# Autodesk Inventor assembly: Shooter
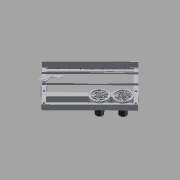
[picture p0: Inventor's stored thumbnail of the model, 180x180]
Saved by Autodesk Inventor 2013 (Build 170138000, 138)
## iProperties
Created: 2013-01-27
Part Number: Shooter
Document SubType Name: Assembly
Designer: Naphat
Author: Naphat
## Documents named in this file (19)
- C:\Autodesk\gruntmaster6000-cad\Shooter6000-cad\Shooter\Shooter.iam
- C:\Autodesk\gruntmaster6000-cad\Shooter6000-cad\Shooter\Basic Wheel\Shooter Basic Design.iam
- C:\Autodesk\gruntmaster6000-cad\Shooter6000-cad\Shooter\26in Angle Channel.ipt
- C:\Autodesk\gruntmaster6000-cad\Shooter6000-cad\Shooter\26in mini C-Channel (rail).ipt
- C:\Users\Naphat\Documents\Inventor\Content Center Files\R2013\en-US\ANSI B18.3(05)\ANSI B18.3 - 1_4-20 UNC - 1(31).ipt
- C:\Users\Naphat\Documents\Inventor\Content Center Files\R2013\en-US\ASTM F436(1)\ASTM F436 - 1_4(1).ipt
- C:\Users\Naphat\Documents\Inventor\Content Center Files\R2013\en-US\IFI 100 107(2)\IFI 100_107 - 1_4 - 20 Metal Type.ipt
- C:\Autodesk\gruntmaster6000-cad\Shooter6000-cad\Shooter\18in C-Channel Front.ipt
- C:\Autodesk\gruntmaster6000-cad\Shooter6000-cad\Shooter\18in C-Channel Rear.ipt
- C:\Users\Naphat\Documents\Inventor\Content Center Files\R2013\en-US\ANSI B18.3(05)\ANSI B18.3 - 1_4-20 UNC - 1.75(31).ipt
- C:\Autodesk\gruntmaster6000-cad\Shooter6000-cad\Shooter\26in Angle Channel CIM Mount Left.ipt
- C:\Autodesk\gruntmaster6000-cad\Shooter6000-cad\Shooter\26in Angle Channel CIM Mount Right.ipt
- C:\Autodesk\gruntmaster6000-cad\Shooter6000-cad\Shooter\26in C-Channel Left.ipt
- C:\Autodesk\gruntmaster6000-cad\Shooter6000-cad\Shooter\26in C-Channel Right.ipt
- C:\Autodesk\gruntmaster6000-cad\Shooter6000-cad\Shooter\Motors\CIM Case\CIM Mount Bolt.ipt
- C:\Autodesk\gruntmaster6000-cad\Shooter6000-cad\Shooter\Firing Pin\Firing Pin.iam
- C:\Autodesk\gruntmaster6000-cad\Shooter6000-cad\Shooter\Frisbee.ipt
- C:\Autodesk\gruntmaster6000-cad\Shooter6000-cad\Imported Components\PG27\PG27.ipt
- C:\Users\Naphat\Documents\Inventor\Content Center Files\R2013\en-US\IFI 100 107(2)\IFI 100_107 - 1_4 - 20 Top Insert Type.ipt
## Components (62 placed, 18 different names)
1. Shooter Basic Design:1 [sub-assembly] — Insert:2, Insert:3
2. Shooter Basic Design:2 [sub-assembly] — Insert:4, Insert:5
3. 26in C-Channel Right:1 — Flush:3, Mate:1, Mate:2, Mate:5, Mate:7, Flush:5, Mate:156, Insert:6, Insert:7, Insert:16, Mate:220, Mate:221
4. 18in C-Channel Rear — Flush:3, Mate:1, Mate:2, Flush:4, Mate:3, Mate:4, Flush:9, Mate:82, Mate:207, Mate:208, Mate:212, Mate:214, Insert:8
5. 18in C-Channel Front — Mate:5, Mate:6, Mate:7, Flush:5, Flush:12, Mate:23, Flush:13, Mate:24, Flush:14, Mate:74, Mate:213, Insert:13
6. 26in C-Channel Left:1 — Flush:4, Mate:3, Mate:4, Mate:6, Mate:8, Mate:9, Mate:75, Mate:76, Mate:77, Mate:78, Mate:79, Mate:80, Mate:81
7. 26in Angle Channel:1 — Mate:8, Mate:9, Flush:9, Mate:25, Mate:36, Mate:38, Mate:39, Mate:40, Mate:41, Mate:42, Mate:43, Mate:44, Mate:45, Mate:46, Mate:47, Mate:48, Mate:49, Mate:50, Mate:51, Mate:52, Mate:53, Mate:54, Mate:55, Mate:56, Mate:57, Mate:58, Mate:59, Mate:60, Mate:61, Mate:62, Mate:63
8. 26in Angle Channel CIM Mount Right:1 — Mate:189, Mate:190, Mate:191, Mate:192, Mate:193, Mate:194, Mate:195, Mate:196, Insert:6, Insert:7, Mate:216, Mate:217, Mate:218, Mate:219
9. 26in Angle Channel CIM Mount Left:3 — Flush:12, Mate:213, Mate:214, Insert:9, Insert:12
10. 26in mini C-Channel (rail):1 — Mate:23, Flush:13, Mate:26, Mate:206
11. 26in mini C-Channel (rail):2 — Mate:24, Flush:14, Mate:25, Mate:26
12. CIM Mount Bolt:1 — Mate:192, Mate:196, Insert:4
13. CIM Mount Bolt:2 — Mate:191, Mate:195, Insert:5
14. CIM Mount Bolt:3 — Mate:189, Mate:193, Insert:2
15. CIM Mount Bolt:4 — Mate:190, Mate:194, Insert:3
16. Firing Pin:1 [sub-assembly] — Mate:207, Mate:208, Mate:210, Mate:211
17. Frisbee:1 — Mate:206
18. PG27:1 — Mate:210, Mate:211, Mate:212
19. Circular Washer (Inch) 1/4:29 — Insert:8, Insert:10
20. Circular Washer (Inch) 1/4:30 — Insert:9, Insert:11
21. Hexagon Socket Head Cap Screw - Inch 1/4 - 20 UNC - 1 3/4:1 — Insert:10, Mate:215
22. Prevailing Torque Type Hex Nut - Inch (IFI) 1/4 - 20 Top Insert Type:1 — Insert:11, Mate:215
23. Circular Washer (Inch) 1/4:31 — Insert:12, Insert:15
24. Circular Washer (Inch) 1/4:32 — Insert:13, Insert:14
25. Hexagon Socket Head Cap Screw - Inch 1/4 - 20 UNC - 1 3/4:2 — Insert:14
26. Prevailing Torque Type Hex Nut - Inch (IFI) 1/4 - 20 Top Insert Type:2 — Insert:15
27. Circular Washer (Inch) 1/4:33 — Insert:16, Mate:222, Mate:223
28. Circular Washer (Inch) 1/4:34 — Mate:216, Mate:217, Mate:226
29. Circular Washer (Inch) 1/4:35 — Mate:218, Mate:219, Mate:228
30. Circular Washer (Inch) 1/4:36 — Mate:220, Mate:221, Mate:224, Mate:225
31. Hexagon Socket Head Cap Screw - Inch 1/4 - 20 UNC - 1 3/4:3 — Mate:224, Mate:225, Mate:229
32. Hexagon Socket Head Cap Screw - Inch 1/4 - 20 UNC - 1 3/4:4 — Mate:222, Mate:223, Mate:227
33. Prevailing Torque Type Hex Nut - Inch (IFI) 1/4 - 20 Top Insert Type:3 — Mate:228, Mate:229
34. Prevailing Torque Type Hex Nut - Inch (IFI) 1/4 - 20 Top Insert Type:4 — Mate:226, Mate:227
35. Hexagon Socket Head Cap Screw - Inch 1/4 - 20 UNC - 1:1 — Mate:36, Mate:72, Mate:91
36. Hexagon Socket Head Cap Screw - Inch 1/4 - 20 UNC - 1:3 — Mate:39, Mate:70, Mate:89
37. Hexagon Socket Head Cap Screw - Inch 1/4 - 20 UNC - 1:4 — Mate:38, Mate:71, Mate:90
38. Hexagon Socket Head Cap Screw - Inch 1/4 - 20 UNC - 1:10 — Mate:43, Mate:66, Mate:85
39. Hexagon Socket Head Cap Screw - Inch 1/4 - 20 UNC - 1:11 — Mate:40, Mate:69, Mate:88
40. Hexagon Socket Head Cap Screw - Inch 1/4 - 20 UNC - 1:14 — Mate:42, Mate:67, Mate:86
41. Hexagon Socket Head Cap Screw - Inch 1/4 - 20 UNC - 1:16 — Mate:44, Mate:65, Mate:84
42. Hexagon Socket Head Cap Screw - Inch 1/4 - 20 UNC - 1:18 — Mate:45, Mate:64, Mate:83
43. Hexagon Socket Head Cap Screw - Inch 1/4 - 20 UNC - 1:22 — Mate:41, Mate:68, Mate:87
44. Prevailing Torque Type Hex Nut - Inch (IFI) 1/4 - 20 Metal Type:2 — Mate:78, Mate:87
45. Prevailing Torque Type Hex Nut - Inch (IFI) 1/4 - 20 Metal Type:8 — Mate:80, Mate:85
46. Prevailing Torque Type Hex Nut - Inch (IFI) 1/4 - 20 Metal Type:9 — Mate:77, Mate:88
47. Prevailing Torque Type Hex Nut - Inch (IFI) 1/4 - 20 Metal Type:14 — Mate:82, Mate:83
48. Prevailing Torque Type Hex Nut - Inch (IFI) 1/4 - 20 Metal Type:24 — Mate:81, Mate:84
49. Prevailing Torque Type Hex Nut - Inch (IFI) 1/4 - 20 Metal Type:27 — Mate:156
50. Prevailing Torque Type Hex Nut - Inch (IFI) 1/4 - 20 Metal Type:41 — Mate:75, Mate:90
51. Prevailing Torque Type Hex Nut - Inch (IFI) 1/4 - 20 Metal Type:42 — Mate:76, Mate:89
52. Prevailing Torque Type Hex Nut - Inch (IFI) 1/4 - 20 Metal Type:43 — Mate:74, Mate:91
53. Prevailing Torque Type Hex Nut - Inch (IFI) 1/4 - 20 Metal Type:48 — Mate:79, Mate:86
54. Circular Washer (Inch) 1/4:1 — Mate:48, Mate:57, Mate:70
55. Circular Washer (Inch) 1/4:2 — Mate:49, Mate:58, Mate:69
56. Circular Washer (Inch) 1/4:3 — Mate:47, Mate:56, Mate:71
57. Circular Washer (Inch) 1/4:4 — Mate:46, Mate:55, Mate:72
58. Circular Washer (Inch) 1/4:7 — Mate:52, Mate:61, Mate:66
59. Circular Washer (Inch) 1/4:8 — Mate:54, Mate:63, Mate:64
60. Circular Washer (Inch) 1/4:9 — Mate:51, Mate:60, Mate:67
61. Circular Washer (Inch) 1/4:10 — Mate:53, Mate:62, Mate:65
62. Circular Washer (Inch) 1/4:28 — Mate:50, Mate:59, Mate:68
## Relationships (121: Mate 99, Insert 15, Flush 7)
- Flush:3: 26in C-Channel Right:1 ↔ 18in C-Channel Rear
- Mate:1: 26in C-Channel Right:1 ↔ 18in C-Channel Rear
- Mate:2: 26in C-Channel Right:1 ↔ 18in C-Channel Rear
- Flush:4: 18in C-Channel Rear ↔ 26in C-Channel Left:1
- Mate:3: 18in C-Channel Rear ↔ 26in C-Channel Left:1
- Mate:4: 18in C-Channel Rear ↔ 26in C-Channel Left:1
- Mate:5: 26in C-Channel Right:1 ↔ 18in C-Channel Front
- Mate:6: 18in C-Channel Front ↔ 26in C-Channel Left:1
- Mate:7: 26in C-Channel Right:1 ↔ 18in C-Channel Front
- Flush:5: 26in C-Channel Right:1 ↔ 18in C-Channel Front
- Mate:8 (-25 mm): 26in C-Channel Left:1 ↔ 26in Angle Channel:1
- Mate:9: 26in C-Channel Left:1 ↔ 26in Angle Channel:1
- Flush:9: 18in C-Channel Rear ↔ 26in Angle Channel:1
- Flush:12: 18in C-Channel Front ↔ 26in Angle Channel CIM Mount Left:3
- Mate:23: 18in C-Channel Front ↔ 26in mini C-Channel (rail):1
- Flush:13: 18in C-Channel Front ↔ 26in mini C-Channel (rail):1
- Mate:24: 18in C-Channel Front ↔ 26in mini C-Channel (rail):2
- Flush:14: 18in C-Channel Front ↔ 26in mini C-Channel (rail):2
- Mate:25 (69.75 mm): 26in Angle Channel:1 ↔ 26in mini C-Channel (rail):2
- Mate:26 (129.5 mm): 26in mini C-Channel (rail):1 ↔ 26in mini C-Channel (rail):2
- Mate:36: 26in Angle Channel:1 ↔ Hexagon Socket Head Cap Screw - Inch 1/4 - 20 UNC - 1:1
- Mate:38: 26in Angle Channel:1 ↔ Hexagon Socket Head Cap Screw - Inch 1/4 - 20 UNC - 1:4
- Mate:39: 26in Angle Channel:1 ↔ Hexagon Socket Head Cap Screw - Inch 1/4 - 20 UNC - 1:3
- Mate:40: 26in Angle Channel:1 ↔ Hexagon Socket Head Cap Screw - Inch 1/4 - 20 UNC - 1:11
- Mate:41: 26in Angle Channel:1 ↔ Hexagon Socket Head Cap Screw - Inch 1/4 - 20 UNC - 1:22
- Mate:42: 26in Angle Channel:1 ↔ Hexagon Socket Head Cap Screw - Inch 1/4 - 20 UNC - 1:14
- Mate:43: 26in Angle Channel:1 ↔ Hexagon Socket Head Cap Screw - Inch 1/4 - 20 UNC - 1:10
- Mate:44: 26in Angle Channel:1 ↔ Hexagon Socket Head Cap Screw - Inch 1/4 - 20 UNC - 1:16
- Mate:45: 26in Angle Channel:1 ↔ Hexagon Socket Head Cap Screw - Inch 1/4 - 20 UNC - 1:18
- Mate:46: 26in Angle Channel:1 ↔ Circular Washer (Inch) 1/4:4
- Mate:47: 26in Angle Channel:1 ↔ Circular Washer (Inch) 1/4:3
- Mate:48: 26in Angle Channel:1 ↔ Circular Washer (Inch) 1/4:1
- Mate:49: 26in Angle Channel:1 ↔ Circular Washer (Inch) 1/4:2
- Mate:50: 26in Angle Channel:1 ↔ Circular Washer (Inch) 1/4:28
- Mate:51: 26in Angle Channel:1 ↔ Circular Washer (Inch) 1/4:9
- Mate:52: 26in Angle Channel:1 ↔ Circular Washer (Inch) 1/4:7
- Mate:53: 26in Angle Channel:1 ↔ Circular Washer (Inch) 1/4:10
- Mate:54: 26in Angle Channel:1 ↔ Circular Washer (Inch) 1/4:8
- Mate:55: 26in Angle Channel:1 ↔ Circular Washer (Inch) 1/4:4
- Mate:56: 26in Angle Channel:1 ↔ Circular Washer (Inch) 1/4:3
- Mate:57: 26in Angle Channel:1 ↔ Circular Washer (Inch) 1/4:1
- Mate:58: 26in Angle Channel:1 ↔ Circular Washer (Inch) 1/4:2
- Mate:59: 26in Angle Channel:1 ↔ Circular Washer (Inch) 1/4:28
- Mate:60: 26in Angle Channel:1 ↔ Circular Washer (Inch) 1/4:9
- Mate:61: 26in Angle Channel:1 ↔ Circular Washer (Inch) 1/4:7
- Mate:62: 26in Angle Channel:1 ↔ Circular Washer (Inch) 1/4:10
- Mate:63: 26in Angle Channel:1 ↔ Circular Washer (Inch) 1/4:8
- Mate:64: Hexagon Socket Head Cap Screw - Inch 1/4 - 20 UNC - 1:18 ↔ Circular Washer (Inch) 1/4:8
- Mate:65: Hexagon Socket Head Cap Screw - Inch 1/4 - 20 UNC - 1:16 ↔ Circular Washer (Inch) 1/4:10
- Mate:66: Hexagon Socket Head Cap Screw - Inch 1/4 - 20 UNC - 1:10 ↔ Circular Washer (Inch) 1/4:7
- Mate:67: Hexagon Socket Head Cap Screw - Inch 1/4 - 20 UNC - 1:14 ↔ Circular Washer (Inch) 1/4:9
- Mate:68: Hexagon Socket Head Cap Screw - Inch 1/4 - 20 UNC - 1:22 ↔ Circular Washer (Inch) 1/4:28
- Mate:69: Hexagon Socket Head Cap Screw - Inch 1/4 - 20 UNC - 1:11 ↔ Circular Washer (Inch) 1/4:2
- Mate:70: Hexagon Socket Head Cap Screw - Inch 1/4 - 20 UNC - 1:3 ↔ Circular Washer (Inch) 1/4:1
- Mate:71: Hexagon Socket Head Cap Screw - Inch 1/4 - 20 UNC - 1:4 ↔ Circular Washer (Inch) 1/4:3
- Mate:72: Hexagon Socket Head Cap Screw - Inch 1/4 - 20 UNC - 1:1 ↔ Circular Washer (Inch) 1/4:4
- Mate:74: 18in C-Channel Front ↔ Prevailing Torque Type Hex Nut - Inch (IFI) 1/4 - 20 Metal Type:43
- Mate:75: 26in C-Channel Left:1 ↔ Prevailing Torque Type Hex Nut - Inch (IFI) 1/4 - 20 Metal Type:41
- Mate:76: 26in C-Channel Left:1 ↔ Prevailing Torque Type Hex Nut - Inch (IFI) 1/4 - 20 Metal Type:42
- Mate:77: 26in C-Channel Left:1 ↔ Prevailing Torque Type Hex Nut - Inch (IFI) 1/4 - 20 Metal Type:9
- Mate:78: 26in C-Channel Left:1 ↔ Prevailing Torque Type Hex Nut - Inch (IFI) 1/4 - 20 Metal Type:2
- Mate:79: 26in C-Channel Left:1 ↔ Prevailing Torque Type Hex Nut - Inch (IFI) 1/4 - 20 Metal Type:48
- Mate:80: 26in C-Channel Left:1 ↔ Prevailing Torque Type Hex Nut - Inch (IFI) 1/4 - 20 Metal Type:8
- Mate:81: 26in C-Channel Left:1 ↔ Prevailing Torque Type Hex Nut - Inch (IFI) 1/4 - 20 Metal Type:24
- Mate:82: 18in C-Channel Rear ↔ Prevailing Torque Type Hex Nut - Inch (IFI) 1/4 - 20 Metal Type:14
- Mate:83: Hexagon Socket Head Cap Screw - Inch 1/4 - 20 UNC - 1:18 ↔ Prevailing Torque Type Hex Nut - Inch (IFI) 1/4 - 20 Metal Type:14
- Mate:84: Hexagon Socket Head Cap Screw - Inch 1/4 - 20 UNC - 1:16 ↔ Prevailing Torque Type Hex Nut - Inch (IFI) 1/4 - 20 Metal Type:24
- Mate:85: Hexagon Socket Head Cap Screw - Inch 1/4 - 20 UNC - 1:10 ↔ Prevailing Torque Type Hex Nut - Inch (IFI) 1/4 - 20 Metal Type:8
- Mate:86: Hexagon Socket Head Cap Screw - Inch 1/4 - 20 UNC - 1:14 ↔ Prevailing Torque Type Hex Nut - Inch (IFI) 1/4 - 20 Metal Type:48
- Mate:87: Hexagon Socket Head Cap Screw - Inch 1/4 - 20 UNC - 1:22 ↔ Prevailing Torque Type Hex Nut - Inch (IFI) 1/4 - 20 Metal Type:2
- Mate:88: Hexagon Socket Head Cap Screw - Inch 1/4 - 20 UNC - 1:11 ↔ Prevailing Torque Type Hex Nut - Inch (IFI) 1/4 - 20 Metal Type:9
- Mate:89: Hexagon Socket Head Cap Screw - Inch 1/4 - 20 UNC - 1:3 ↔ Prevailing Torque Type Hex Nut - Inch (IFI) 1/4 - 20 Metal Type:42
- Mate:90: Hexagon Socket Head Cap Screw - Inch 1/4 - 20 UNC - 1:4 ↔ Prevailing Torque Type Hex Nut - Inch (IFI) 1/4 - 20 Metal Type:41
- Mate:91: Hexagon Socket Head Cap Screw - Inch 1/4 - 20 UNC - 1:1 ↔ Prevailing Torque Type Hex Nut - Inch (IFI) 1/4 - 20 Metal Type:43
- Mate:156: 26in C-Channel Right:1 ↔ Prevailing Torque Type Hex Nut - Inch (IFI) 1/4 - 20 Metal Type:27
- Mate:189: 26in Angle Channel CIM Mount Right:1 ↔ CIM Mount Bolt:3
- Mate:190: 26in Angle Channel CIM Mount Right:1 ↔ CIM Mount Bolt:4
- Mate:191: 26in Angle Channel CIM Mount Right:1 ↔ CIM Mount Bolt:2
- Mate:192: 26in Angle Channel CIM Mount Right:1 ↔ CIM Mount Bolt:1
- Mate:193: 26in Angle Channel CIM Mount Right:1 ↔ CIM Mount Bolt:3
- Mate:194: 26in Angle Channel CIM Mount Right:1 ↔ CIM Mount Bolt:4
- Mate:195: 26in Angle Channel CIM Mount Right:1 ↔ CIM Mount Bolt:2
- Mate:196: 26in Angle Channel CIM Mount Right:1 ↔ CIM Mount Bolt:1
- Mate:206: 26in mini C-Channel (rail):1 ↔ Frisbee:1
- Mate:207: 18in C-Channel Rear ↔ Firing Pin:1
- Mate:208: 18in C-Channel Rear ↔ Firing Pin:1
- Mate:210: Firing Pin:1 ↔ PG27:1
- Mate:211: Firing Pin:1 ↔ PG27:1
- Mate:212: 18in C-Channel Rear ↔ PG27:1
- Insert:2: Shooter Basic Design:1 ↔ CIM Mount Bolt:3
- Insert:3: Shooter Basic Design:1 ↔ CIM Mount Bolt:4
- Insert:4: Shooter Basic Design:2 ↔ CIM Mount Bolt:1
- Insert:5: Shooter Basic Design:2 ↔ CIM Mount Bolt:2
- Insert:6: 26in C-Channel Right:1 ↔ 26in Angle Channel CIM Mount Right:1
- Insert:7: 26in C-Channel Right:1 ↔ 26in Angle Channel CIM Mount Right:1
- Mate:213: 18in C-Channel Front ↔ 26in Angle Channel CIM Mount Left:3
- Mate:214: 18in C-Channel Rear ↔ 26in Angle Channel CIM Mount Left:3
- Mate:215: Hexagon Socket Head Cap Screw - Inch 1/4 - 20 UNC - 1 3/4:1 ↔ Prevailing Torque Type Hex Nut - Inch (IFI) 1/4 - 20 Top Insert Type:1
- Mate:216: 26in Angle Channel CIM Mount Right:1 ↔ Circular Washer (Inch) 1/4:34
- Mate:217: 26in Angle Channel CIM Mount Right:1 ↔ Circular Washer (Inch) 1/4:34
- Mate:218: 26in Angle Channel CIM Mount Right:1 ↔ Circular Washer (Inch) 1/4:35
- Mate:219: 26in Angle Channel CIM Mount Right:1 ↔ Circular Washer (Inch) 1/4:35
- Mate:220: 26in C-Channel Right:1 ↔ Circular Washer (Inch) 1/4:36
- Mate:221: 26in C-Channel Right:1 ↔ Circular Washer (Inch) 1/4:36
- Mate:222: Circular Washer (Inch) 1/4:33 ↔ Hexagon Socket Head Cap Screw - Inch 1/4 - 20 UNC - 1 3/4:4
- Mate:223: Circular Washer (Inch) 1/4:33 ↔ Hexagon Socket Head Cap Screw - Inch 1/4 - 20 UNC - 1 3/4:4
- Mate:224: Circular Washer (Inch) 1/4:36 ↔ Hexagon Socket Head Cap Screw - Inch 1/4 - 20 UNC - 1 3/4:3
- Mate:225: Circular Washer (Inch) 1/4:36 ↔ Hexagon Socket Head Cap Screw - Inch 1/4 - 20 UNC - 1 3/4:3
- Mate:226: Circular Washer (Inch) 1/4:34 ↔ Prevailing Torque Type Hex Nut - Inch (IFI) 1/4 - 20 Top Insert Type:4
- Mate:227: Hexagon Socket Head Cap Screw - Inch 1/4 - 20 UNC - 1 3/4:4 ↔ Prevailing Torque Type Hex Nut - Inch (IFI) 1/4 - 20 Top Insert Type:4
- Mate:228: Circular Washer (Inch) 1/4:35 ↔ Prevailing Torque Type Hex Nut - Inch (IFI) 1/4 - 20 Top Insert Type:3
- Mate:229: Hexagon Socket Head Cap Screw - Inch 1/4 - 20 UNC - 1 3/4:3 ↔ Prevailing Torque Type Hex Nut - Inch (IFI) 1/4 - 20 Top Insert Type:3
- Insert:8: 18in C-Channel Rear ↔ Circular Washer (Inch) 1/4:29
- Insert:9: 26in Angle Channel CIM Mount Left:3 ↔ Circular Washer (Inch) 1/4:30
- Insert:10: Circular Washer (Inch) 1/4:29 ↔ Hexagon Socket Head Cap Screw - Inch 1/4 - 20 UNC - 1 3/4:1
- Insert:11: Circular Washer (Inch) 1/4:30 ↔ Prevailing Torque Type Hex Nut - Inch (IFI) 1/4 - 20 Top Insert Type:1
- Insert:12: 26in Angle Channel CIM Mount Left:3 ↔ Circular Washer (Inch) 1/4:31
- Insert:13: 18in C-Channel Front ↔ Circular Washer (Inch) 1/4:32
- Insert:14: Circular Washer (Inch) 1/4:32 ↔ Hexagon Socket Head Cap Screw - Inch 1/4 - 20 UNC - 1 3/4:2
- Insert:15: Circular Washer (Inch) 1/4:31 ↔ Prevailing Torque Type Hex Nut - Inch (IFI) 1/4 - 20 Top Insert Type:2
- Insert:16: 26in C-Channel Right:1 ↔ Circular Washer (Inch) 1/4:33
